# Autodesk Inventor assembly: MainAssy
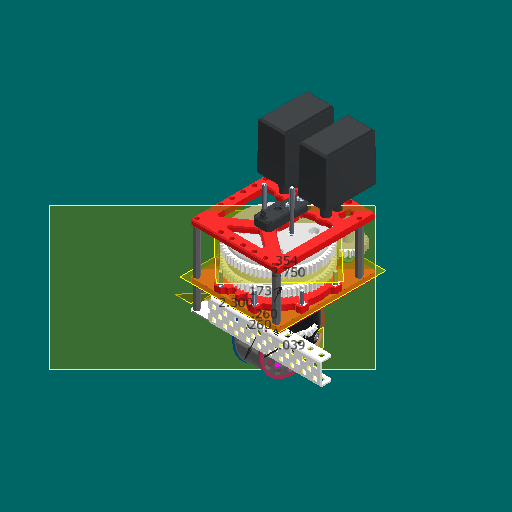
[picture p0: Inventor's stored thumbnail of the model, 512x512]
Saved by Autodesk Inventor 2023.1 (Build 271208000, 208)
## iProperties
Created: 2022-10-29
Part Number: MainAssy
Document SubType Name: Assembly
Designer: zac-h
Author: zac-h
## iProperties of the stored document 0.188 ID x 0.500 OD x 0.196 WD (Radial Bearing) (217-3246).ipt
Created: 2013-12-06
Part Number: 217-3246-STEP
Material: Generic
Description: STEP AP214
Document SubType Name: Modeling
Designer: zac-h
Density: 1 g/cm^3
Appearance: Default
Sending System: SolidWorks 2013
Preprocessor: SwSTEP 2.0
Title: 217-3246-STEP.STEP
Revision Number: ANY
## Documents named in this file (42)
- C:\Users\zac-h\Documents\CAD\guardSwerve5\MainAssy.iam
- C:\Users\zac-h\Documents\CAD\guardSwerve5\WheelHalf.ipt
- C:\Users\zac-h\Documents\CAD\guardSwerve5\WheelHalf_MIR.ipt
- C:\Users\zac-h\Documents\CAD\guardSwerve5\Carriage.ipt
- C:\Users\zac-h\Documents\CAD\guardSwerve5\MainAssy\Design Accelerator\Bevel Gears1.iam
- **C:\Users\zac-h\Documents\CAD\guardSwerve5\MainAssy.iam*LocalDocs*xAaaaa1caAaaaaaaaAaaaqx3fTa*0.188 ID x 0.500 OD x 0.196 WD (Radial Bearing) (217-3246).ipt
- C:\Users\zac-h\Documents\CAD\VEX-CAD-Inventor-1.3.0\VEX-CAD-Inventor-1.3.0\Motion\Circle Insert.ipt
- C:\Users\zac-h\Documents\CAD\guardSwerve5\608bearing.ipt
- C:\Users\zac-h\Documents\CAD\guardSwerve1\bearingsleeve.ipt
- C:\Users\zac-h\Documents\CAD\VEX-CAD-Inventor-1.3.0\VEX-CAD-Inventor-1.3.0\Structure\Hardware\Screw Steel - Star\SScrew Star Smooth .500.ipt
- C:\Users\zac-h\Documents\CAD\VEX-CAD-Inventor-1.3.0\VEX-CAD-Inventor-1.3.0\Structure\Hardware\Screw Steel - Star\SScrew Star Smooth .250.ipt
- C:\Users\zac-h\Documents\CAD\guardSwerve5\Baseplate.ipt
- C:\Users\zac-h\Documents\CAD\VEX-CAD-Inventor-1.3.0\VEX-CAD-Inventor-1.3.0\Structure\C-Channels\Aluminum 1x2x1\Alu C 1x2x1x10.ipt
- C:\Users\zac-h\Documents\CAD\guardSwerve5\UpperRaceRing.ipt
- C:\Users\zac-h\Documents\CAD\guardSwerve5\SteeringCoupler.ipt
- C:\Users\zac-h\Documents\CAD\guardSwerve5\MainAssy\Design Accelerator\Spur Gears1.iam
- C:\Users\zac-h\Documents\CAD\guardSwerve5\MainAssy\Design Accelerator\Spur Gears2.iam
- C:\Users\zac-h\Documents\CAD\guardSwerve5\MainAssy\Design Accelerator\Spur Gears4.iam
- C:\Users\zac-h\Documents\CAD\guardSwerve5\MainAssy\Design Accelerator\Spur Gears5.iam
- C:\Users\zac-h\Documents\CAD\guardSwerve5\MainAssy\Design Accelerator\Spur Gears3.iam
- C:\Users\zac-h\Documents\CAD\guardSwerve5\MainAssy\Design Accelerator\Spur Gears6.iam
- C:\Users\zac-h\Documents\CAD\guardSwerve5\UpperRingSeat.ipt
- C:\Users\zac-h\Documents\CAD\VEX-CAD-Inventor-1.3.0\VEX-CAD-Inventor-1.3.0\Structure\Hardware\Screw Steel - Star\SScrew Star Smooth 1.000.ipt
- C:\Users\zac-h\Documents\CAD\guardSwerve5\DiffCap.ipt
- C:\Users\zac-h\Documents\CAD\VEX-CAD-Inventor-1.3.0\VEX-CAD-Inventor-1.3.0\Motion\Square Insert.ipt
- C:\Users\zac-h\Documents\CAD\VEX-CAD-Inventor-1.3.0\VEX-CAD-Inventor-1.3.0\Structure\Hardware\Screw Steel - Star\SScrew Star Smooth .875.ipt
- C:\Users\zac-h\Documents\CAD\VEX-CAD-Inventor-1.3.0\VEX-CAD-Inventor-1.3.0\Structure\Hardware\Nut Nylock.ipt
- C:\Users\zac-h\Documents\CAD\VEX-CAD-Inventor-1.3.0\VEX-CAD-Inventor-1.3.0\Structure\Hardware\Screw Steel - Star\SScrew Star Smooth 1.750.ipt
- C:\Users\zac-h\Documents\CAD\VEX-CAD-Inventor-1.3.0\VEX-CAD-Inventor-1.3.0\Structure\Hardware\Screw Steel - Star\SScrew Star Smooth 1.250.ipt
- C:\Users\zac-h\Documents\CAD\VEX-CAD-Inventor-1.3.0\VEX-CAD-Inventor-1.3.0\Motion\Shaft LS\Shaft LS 3.0 in.ipt
- C:\Users\zac-h\Documents\CAD\VEX-CAD-Inventor-1.3.0\VEX-CAD-Inventor-1.3.0\Structure\Standoff\Standoff 2.00.ipt
- C:\Users\zac-h\Documents\CAD\guardSwerve5\TopPlate.ipt
- C:\Users\zac-h\Documents\CAD\VEX-CAD-Inventor-1.3.0\VEX-CAD-Inventor-1.3.0\Electronics\V5 Simple Motor.ipt
- C:\Users\zac-h\Documents\CAD\VEX-CAD-Inventor-1.3.0\VEX-CAD-Inventor-1.3.0\Electronics\Sensors\Potentiometer V2.ipt
- C:\Users\zac-h\Documents\CAD\VEX-CAD-Inventor-1.3.0\VEX-CAD-Inventor-1.3.0\Structure\Hardware\Screw Steel - Star\SScrew Star Smooth .750.ipt
- C:\Users\zac-h\Documents\CAD\guardSwerve5\UnderGusset.ipt
- C:\Users\zac-h\Documents\CAD\VEX-CAD-Inventor-1.3.0\VEX-CAD-Inventor-1.3.0\Structure\Standoff\Standoff 1.00.ipt
- C:\Users\zac-h\Documents\CAD\guardSwerve5\1.2inSpacer.ipt
- C:\Users\Zac Hah\Documents\GitHub\spin-up-cad\VEX-CAD-Inventor-1.3.0\VEX-CAD-Inventor-1.3.0\Structure\Hardware\Screw Steel - Star.ipt
- C:\Users\Zac Hah\Documents\GitHub\spin-up-cad\VEX-CAD-Inventor-1.3.0\VEX-CAD-Inventor-1.3.0\Motion\Shaft LS.ipt
- C:\Users\Zac Hah\Documents\GitHub\spin-up-cad\VEX-CAD-Inventor-1.3.0\VEX-CAD-Inventor-1.3.0\Structure\Standoff.ipt
- C:\Users\zac-h\Documents\CAD\VEX-CAD-Inventor-1.3.0\VEX-CAD-Inventor-1.3.0\Motion\0.188 ID x 0.500 OD x 0.196 WD (Radial Bearing) (217-3246).step
## Components (86 placed, 33 different names)
1. WheelHalf:1 — Mate:1
2. WheelHalf_MIR:1 — Flush:1, Mate:25, Angle:5
3. Carriage:1 — Flush:1, Mate:4, Mate:5, Mate:6, Mate:7, Insert:1, Insert:3, Insert:10, Insert:11, Insert:12, Flush:2, Insert:36, Insert:37, Insert:38, Insert:39, Mate:24, Angle:4
4. Bevel Gears:1 [sub-assembly] — Mate:1, Mate:4, Insert:59, Mate:24, Angle:4, Mate:25, Angle:5
5. 0.188 ID x 0.500 OD x 0.196 WD (Radial Bearing) (217-3246):1 — Insert:10
6. 0.188 ID x 0.500 OD x 0.196 WD (Radial Bearing) (217-3246):2 — Insert:1
7. Circle Insert:1 — Mate:5, Mate:6, Mate:7
8. Circle Insert:4 — Insert:49
9. Circle Insert:5 — Insert:44
10. Baseplate:1 — Flush:2, Insert:14, Insert:15, Insert:16, Flush:3, Flush:4, Insert:21, Insert:27, Insert:28, Insert:66, Insert:67, Insert:68, Insert:69
11. Alu C 1x2x1x10:1 — Insert:14, Insert:21, Flush:13, Flush:14
12. Alu C 1x2x1x10:2 — Insert:15, Insert:16
13. UpperRaceRing:1 — Flush:3, Flush:4, Insert:29
14. SteeringCoupler:1 — Flush:5, Mate:20, Mate:21, Insert:31, Insert:32, Insert:33, Insert:34, Flush:8, Insert:45, Insert:63, Insert:64, Insert:65
15. Spur Gears:1 [sub-assembly] — Flush:7, Insert:31, Insert:49
16. Spur Gears:2 [sub-assembly] — Insert:30, Mate:20, Mate:21, Mate:23, Flush:11
17. RingGear [sub-assembly] — Insert:30, Mate:23, Flush:11
18. Circle Insert:7 — Insert:28, Insert:85
19. Circle Insert:8 — Insert:27, Mate:15
20. Spur Gears:4 [sub-assembly] — Mate:15, Flush:7, Flush:15
21. Spur Gears:5 [sub-assembly] — Insert:32, Insert:43
22. Spur Gears:6 [sub-assembly] — Insert:33, Insert:44
23. Spur Gears:7 [sub-assembly] — Insert:34, Insert:42
24. UpperRingSeat:1 — Flush:8, Insert:35, Insert:41, Flush:9, Flush:10, Insert:48
25. Spur Gears:8 [sub-assembly] — Insert:35, Insert:51
26. SScrew Star Smooth 1.000:28 — Insert:39
27. SScrew Star Smooth 1.000:29 — Insert:38
28. SScrew Star Smooth 1.000:30 — Insert:37
29. SScrew Star Smooth 1.000:31 — Insert:36
30. RingGear:2 [sub-assembly] — Insert:41
31. DiffCap:1 — Flush:9, Flush:10, Insert:58, Insert:60, Insert:61, Insert:62
32. Square Insert:1 — Insert:42
33. Circle Insert:9 — Insert:43
34. SScrew Star Smooth .875:33 — Insert:45
35. Nut Nylock:1 — Insert:48
36. Circle Insert:10 — Insert:51
37. Shaft LS 3.0 in:1 — Insert:59
38. SScrew Star Smooth 1.750:47 — Insert:62
39. SScrew Star Smooth 1.750:48 — Insert:61
40. SScrew Star Smooth 1.750:49 — Insert:60
41. Nut Nylock:2 — Insert:63
42. Nut Nylock:3 — Insert:64
43. Nut Nylock:4 — Insert:65
44. Standoff 2.00:1 — Insert:69
45. Standoff 2.00:2 — Insert:66
46. Standoff 2.00:3 — Insert:67
47. Standoff 2.00:4 — Insert:68, Flush:12
48. TopPlate:1 — Flush:12, Insert:70, Insert:71, Insert:72, Insert:73, Insert:76, Insert:77, Insert:78, Insert:79, Insert:80
49. V5 Simple Motor:1 — Insert:72, Insert:73
50. V5 Simple Motor:2 — Insert:70, Insert:71
51. Potentiometer V2:1 — Insert:80, Insert:81, Insert:82
52. SScrew Star Smooth .750:50 — Insert:76
53. SScrew Star Smooth .750:51 — Insert:77
54. SScrew Star Smooth .750:52 — Insert:78
55. SScrew Star Smooth .750:53 — Insert:79
56. SScrew Star Smooth .500:54 — Insert:81
57. SScrew Star Smooth .500:55 — Insert:82
58. UnderGusset:1 — Flush:13, Flush:14, Insert:83, Insert:84
59. Standoff 1.00:5 — Insert:83
60. SScrew Star Smooth .500:56 — Insert:84
61. 1.2inSpacer:1 — Flush:15
62. Spur Gears:10 [sub-assembly] — Insert:85
63. SScrew Star Smooth .250:5 — Insert:11
64. SScrew Star Smooth .250:6 — Insert:12
65. SScrew Star Smooth .250:7
66. SScrew Star Smooth .250:8
67. bearingsleeve:1 — Insert:2, Insert:3
68. 608bearing:1 — Insert:2, Flush:5
69. bearingsleeve:2
70. 608bearing:2
71. bearingsleeve:3
72. 608bearing:3
73. bearingsleeve:4
74. 608bearing:4
75. SScrew Star Smooth .500:20 — Insert:29
76. SScrew Star Smooth .500:21
77. SScrew Star Smooth .500:22
78. SScrew Star Smooth .500:23
79. SScrew Star Smooth .500:24
80. SScrew Star Smooth .500:25
81. SScrew Star Smooth .500:26
82. SScrew Star Smooth .500:27
83. SScrew Star Smooth 1.250:40 — Insert:58
84. SScrew Star Smooth 1.250:44
85. SScrew Star Smooth 1.250:45
86. SScrew Star Smooth 1.250:46
## Component patterns: (2 elements, first: SScrew Star Smooth .250:5 + SScrew Star Smooth .250:6), (4 elements, first: bearingsleeve:1 + 608bearing:1), (8 elements, first: SScrew Star Smooth .500:20), (4 elements, first: SScrew Star Smooth 1.250:40)
## Relationships (86: Insert 57, Flush 14, Mate 12, Angle 3)
- Mate:1: WheelHalf:1 ↔ Bevel Gears:1
- Flush:1: WheelHalf_MIR:1 ↔ Carriage:1
- Mate:4: Carriage:1 ↔ Bevel Gears:1
- Mate:5: Carriage:1 ↔ Circle Insert:1
- Mate:6: Carriage:1 ↔ Circle Insert:1
- Mate:7: Carriage:1 ↔ Circle Insert:1
- Insert:1: Carriage:1 ↔ 0.188 ID x 0.500 OD x 0.196 WD (Radial Bearing) (217-3246):2
- Insert:2: bearingsleeve:1 ↔ 608bearing:1
- Insert:3: Carriage:1 ↔ bearingsleeve:1
- Insert:10: Carriage:1 ↔ 0.188 ID x 0.500 OD x 0.196 WD (Radial Bearing) (217-3246):1
- Insert:11: Carriage:1 ↔ SScrew Star Smooth .250:5
- Insert:12: Carriage:1 ↔ SScrew Star Smooth .250:6
- Flush:2: Carriage:1 ↔ Baseplate:1
- Insert:14: Baseplate:1 ↔ Alu C 1x2x1x10:1
- Insert:15: Baseplate:1 ↔ Alu C 1x2x1x10:2
- Insert:16: Baseplate:1 ↔ Alu C 1x2x1x10:2
- Flush:3: Baseplate:1 ↔ UpperRaceRing:1
- Flush:4: Baseplate:1 ↔ UpperRaceRing:1
- Insert:21: Baseplate:1 ↔ Alu C 1x2x1x10:1
- Flush:5: SteeringCoupler:1 ↔ 608bearing:1
- Insert:27: Baseplate:1 ↔ Circle Insert:8
- Insert:28: Baseplate:1 ↔ Circle Insert:7
- Mate:15: Circle Insert:8 ↔ Spur Gears:4
- Flush:7: Spur Gears:1 ↔ Spur Gears:4
- Insert:29: UpperRaceRing:1 ↔ SScrew Star Smooth .500:20
- Insert:30: Spur Gears:2 ↔ RingGear
- Mate:20: SteeringCoupler:1 ↔ Spur Gears:2
- Mate:21: SteeringCoupler:1 ↔ Spur Gears:2
- Insert:31: SteeringCoupler:1 ↔ Spur Gears:1
- Insert:32: SteeringCoupler:1 ↔ Spur Gears:5
- Insert:33: SteeringCoupler:1 ↔ Spur Gears:6
- Insert:34 (1.27 mm): SteeringCoupler:1 ↔ Spur Gears:7
- Flush:8: SteeringCoupler:1 ↔ UpperRingSeat:1
- Insert:35: UpperRingSeat:1 ↔ Spur Gears:8
- Insert:36: Carriage:1 ↔ SScrew Star Smooth 1.000:31
- Insert:37: Carriage:1 ↔ SScrew Star Smooth 1.000:30
- Insert:38: Carriage:1 ↔ SScrew Star Smooth 1.000:29
- Insert:39: Carriage:1 ↔ SScrew Star Smooth 1.000:28
- Insert:41: UpperRingSeat:1 ↔ RingGear:2
- Flush:9: UpperRingSeat:1 ↔ DiffCap:1
- Flush:10: UpperRingSeat:1 ↔ DiffCap:1
- Insert:42: Spur Gears:7 ↔ Square Insert:1
- Insert:43: Spur Gears:5 ↔ Circle Insert:9
- Insert:44: Circle Insert:5 ↔ Spur Gears:6
- Insert:45: SteeringCoupler:1 ↔ SScrew Star Smooth .875:33
- Insert:48: UpperRingSeat:1 ↔ Nut Nylock:1
- Insert:49: Circle Insert:4 ↔ Spur Gears:1
- Insert:51: Spur Gears:8 ↔ Circle Insert:10
- Mate:22
- Angle:3 (45 deg)
- Insert:58: DiffCap:1 ↔ SScrew Star Smooth 1.250:40
- Insert:59: Bevel Gears:1 ↔ Shaft LS 3.0 in:1
- Mate:23: Spur Gears:2 ↔ RingGear
- Flush:11: Spur Gears:2 ↔ RingGear
- Insert:60: DiffCap:1 ↔ SScrew Star Smooth 1.750:49
- Insert:61: DiffCap:1 ↔ SScrew Star Smooth 1.750:48
- Insert:62: DiffCap:1 ↔ SScrew Star Smooth 1.750:47
- Insert:63: SteeringCoupler:1 ↔ Nut Nylock:2
- Insert:64: SteeringCoupler:1 ↔ Nut Nylock:3
- Insert:65: SteeringCoupler:1 ↔ Nut Nylock:4
- Insert:66: Baseplate:1 ↔ Standoff 2.00:2
- Insert:67: Baseplate:1 ↔ Standoff 2.00:3
- Insert:68: Baseplate:1 ↔ Standoff 2.00:4
- Insert:69: Baseplate:1 ↔ Standoff 2.00:1
- Flush:12: Standoff 2.00:4 ↔ TopPlate:1
- Insert:70: TopPlate:1 ↔ V5 Simple Motor:2
- Insert:71: TopPlate:1 ↔ V5 Simple Motor:2
- Insert:72: TopPlate:1 ↔ V5 Simple Motor:1
- Insert:73: TopPlate:1 ↔ V5 Simple Motor:1
- Insert:76: TopPlate:1 ↔ SScrew Star Smooth .750:50
- Insert:77: TopPlate:1 ↔ SScrew Star Smooth .750:51
- Insert:78: TopPlate:1 ↔ SScrew Star Smooth .750:52
- Insert:79: TopPlate:1 ↔ SScrew Star Smooth .750:53
- Insert:80: TopPlate:1 ↔ Potentiometer V2:1
- Insert:81: Potentiometer V2:1 ↔ SScrew Star Smooth .500:54
- Insert:82: Potentiometer V2:1 ↔ SScrew Star Smooth .500:55
- Flush:13: Alu C 1x2x1x10:1 ↔ UnderGusset:1
- Flush:14: Alu C 1x2x1x10:1 ↔ UnderGusset:1
- Insert:83: UnderGusset:1 ↔ Standoff 1.00:5
- Insert:84: UnderGusset:1 ↔ SScrew Star Smooth .500:56
- Flush:15: Spur Gears:4 ↔ 1.2inSpacer:1
- Insert:85 (28.575 mm): Circle Insert:7 ↔ Spur Gears:10
- Mate:24: Carriage:1 ↔ Bevel Gears:1
- Angle:4 (0 deg): Carriage:1 ↔ Bevel Gears:1
- Mate:25: WheelHalf_MIR:1 ↔ Bevel Gears:1
- Angle:5 (0 deg): WheelHalf_MIR:1 ↔ Bevel Gears:1
